# Autodesk Inventor assembly: SMLM_Holder_v1
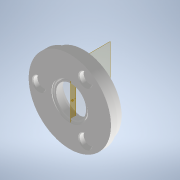
[picture p0: Inventor's stored thumbnail of the model, 180x180]
Saved by Autodesk Inventor 2022 (Build 260153000, 153)
## iProperties
Created: 2021-11-24
Part Number: SMLM_Holder_v1
Material: Generisch
Document SubType Name: Assembly
Designer: Muriel
Author: Muriel
## Documents named in this file (5)
- C:\Users\diederichbenedict\Dropbox\Dokumente\Promotion\PROJECTS\UC2\02_CAD\INVENTOR\uc2_v3\SMLM_Holder\SMLM_Holder_v1.iam
- C:\Users\diederichbenedict\Dropbox\Dokumente\Promotion\PROJECTS\UC2\02_CAD\INVENTOR\uc2_v3\SMLM_Holder\00_Coverglass_25mm.ipt
- C:\Users\diederichbenedict\Dropbox\Dokumente\Promotion\PROJECTS\UC2\02_CAD\INVENTOR\uc2_v3\SMLM_Holder\00_0-ring.ipt
- C:\Users\diederichbenedict\Dropbox\Dokumente\Promotion\PROJECTS\UC2\02_CAD\INVENTOR\uc2_v3\SMLM_Holder\01_SMLM_Holder_Base.ipt
- C:\Users\diederichbenedict\Dropbox\Dokumente\Promotion\PROJECTS\UC2\02_CAD\INVENTOR\uc2_v3\SMLM_Holder\02_SMLM_Holdre_Bottom.ipt
## Components (4 placed, 4 different names)
1. 00_Coverglass_25mm:1 — Passend:1, Tangential:1
2. 00_0-ring:1 — Fluchtend:2, Passend:1, Tangential:1, Passend:2, Passend:3, Winkel:1
3. 01_SMLM_Holder_Base:1 — Fluchtend:3, Fluchtend:4, Fluchtend:5
4. 02_SMLM_Holdre_Bottom:1 — Fluchtend:4, Fluchtend:5
## Relationships (10: Flush 4, Mate 4, Tangent 1, Angle 1)
- Fluchtend:2 [Flush]: 00_0-ring:1
- Passend:1 [Mate]: 00_Coverglass_25mm:1 ↔ 00_0-ring:1
- Tangential:1: 00_Coverglass_25mm:1 ↔ 00_0-ring:1
- Passend:2 [Mate]: 00_0-ring:1
- Passend:3 [Mate]: 00_0-ring:1
- Passend:4 [Mate]
- Winkel:1 [Angle] (0 deg): 00_0-ring:1
- Fluchtend:3 [Flush]: 01_SMLM_Holder_Base:1
- Fluchtend:4 [Flush]: 01_SMLM_Holder_Base:1 ↔ 02_SMLM_Holdre_Bottom:1
- Fluchtend:5 [Flush]: 01_SMLM_Holder_Base:1 ↔ 02_SMLM_Holdre_Bottom:1
